# Autodesk Inventor assembly: ASY ДМФ 0100 Барабан
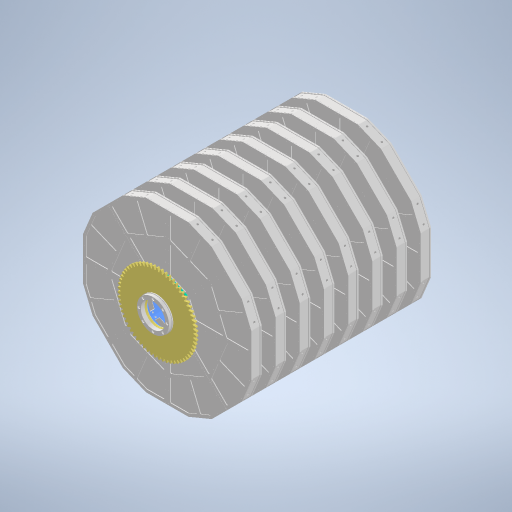
[picture p0: Inventor's stored thumbnail of the model, 512x512]
Saved by Autodesk Inventor 2024.2 (Build 282272000, 272)
## iProperties
Created: 2024-04-28
Part Number: ASY ДМФ 0100 Барабан
Document SubType Name: Assembly
Designer: pokla
Author: pokla
## Documents named in this file (13)
- C:\Users\pokla\Documents\Inventor\ДФО\ДМФ\DMF-Disk-Micro-Filter\ASY ДМФ 0100 Барабан.iam
- C:\Users\pokla\Documents\Inventor\ДФО\ДМФ\DMF-Disk-Micro-Filter\ДМФ 01 21 Барабан торец НОС.ipt
- C:\Users\pokla\Documents\Inventor\ДФО\ДМФ\DMF-Disk-Micro-Filter\ДМФ 01 13 Барабан Лист лев брт.ipt
- C:\Users\pokla\Documents\Inventor\ДФО\ДМФ\DMF-Disk-Micro-Filter\ДМФ 01 14 Барабан Лист прав брт.ipt
- C:\Users\pokla\Documents\Inventor\ДФО\ДМФ\DMF-Disk-Micro-Filter\ДМФ 01 31 Барабан Опорное кольцо НОС.ipt
- C:\Users\pokla\Documents\Inventor\ДФО\ДМФ\DMF-Disk-Micro-Filter\ДМФ 01 17 опора крышки.ipt
- C:\Users\pokla\Documents\Inventor\ДФО\ДМФ\DMF-Disk-Micro-Filter\ДМС 000 размеры.ipt
- C:\Users\pokla\Documents\Inventor\ДФО\ДМФ\DMF-Disk-Micro-Filter\ДМФ 01 41 Шестерня ведомая.ipt
- C:\Users\pokla\Documents\Inventor\ДФО\ДМФ\DMF-Disk-Micro-Filter\ДМФ 01 12 Барабан усилитель.ipt
- C:\Users\pokla\Documents\Inventor\ДФО\ДМФ\DMF-Disk-Micro-Filter\ASY ДМФ 010 крышка.iam
- C:\Users\pokla\Documents\Inventor\ДФО\ДМФ\DMF-Disk-Micro-Filter\ДМФ 01 32 Барабан Опорное кольцо КОРМА.ipt
- C:\Users\pokla\Documents\Inventor\ДФО\ДМФ\DMF-Disk-Micro-Filter\ДМФ 01 22 Барабан торец КОРМА.ipt
- C:\Users\pokla\Documents\Inventor\ДФО\ДМФ\DMF-Disk-Micro-Filter\ASY фильтр пакет.iam
## Components (67 placed, 12 different names)
1. ДМС 000 размеры:1
2. ДМФ 01 21 Барабан торец НОС:2 — Mate:15, Flush:8, Flush:9, Flush:10, Flush:11, Mate:16, Mate:17, Rigid:19, Mate:19, Flush:14, Mate:21, Flush:15, Flush:16, Flush:17, Mate:23
3. ДМФ 01 31 Барабан Опорное кольцо НОС:1 — Rotational:1
4. ДМФ 01 32 Барабан Опорное кольцо КОРМА:1 — Mate:14, Rigid:18
5. ДМФ 01 22 Барабан торец КОРМА:1 — Rigid:18, Flush:12, Flush:13, Mate:18
6. ДМФ 01 13 Барабан Лист лев брт:1 — Mate:12, Flush:7, Flush:10, Flush:11, Mate:16, Flush:13, Mate:18, Mate:20
7. ДМФ 01 14 Барабан Лист прав брт:1 — Mate:11, Flush:8, Flush:9, Mate:17, Flush:12, Mate:22
8. ДМФ 01 17 опора крышки:1 — Mate:21, Flush:15, Mate:22
9. ДМФ 01 17 опора крышки:2 — Mate:19, Mate:20, Flush:14
10. ДМС 105 Шестерня ведомая:1 — Rigid:19, Rotational:1
11. ASY ДМФ 010 крышка:1 [sub-assembly] — Flush:16, Flush:17, Mate:23
12. ДМФ 01 12 Барабан усилитель:4 — Rigid:10
13. ДМФ 01 12 Барабан усилитель:1 — Rigid:8
14. ДМФ 01 12 Барабан усилитель:5 — Rigid:10, Rigid:11, Rigid:14
15. ДМФ 01 12 Барабан усилитель:2 — Rigid:8, Rigid:9, Rigid:14
16. ДМФ 01 12 Барабан усилитель:3 — Rigid:9, Mate:12
17. ДМФ 01 12 Барабан усилитель:6 — Rigid:11
18. ДМФ 01 12 Барабан усилитель:7
19. ДМФ 01 12 Барабан усилитель:8
20. ДМФ 01 12 Барабан усилитель:21
21. ДМФ 01 12 Барабан усилитель:28
22. ДМФ 01 12 Барабан усилитель:35
23. ДМФ 01 12 Барабан усилитель:42
24. ДМФ 01 12 Барабан усилитель:9
25. ДМФ 01 12 Барабан усилитель:10
26. ДМФ 01 12 Барабан усилитель:22
27. ДМФ 01 12 Барабан усилитель:29
28. ДМФ 01 12 Барабан усилитель:36
29. ДМФ 01 12 Барабан усилитель:43
30. ДМФ 01 12 Барабан усилитель:11
31. ДМФ 01 12 Барабан усилитель:12
32. ДМФ 01 12 Барабан усилитель:23
33. ДМФ 01 12 Барабан усилитель:30
34. ДМФ 01 12 Барабан усилитель:37
35. ДМФ 01 12 Барабан усилитель:44
36. ДМФ 01 12 Барабан усилитель:13
37. ДМФ 01 12 Барабан усилитель:14
38. ДМФ 01 12 Барабан усилитель:24
39. ДМФ 01 12 Барабан усилитель:31
40. ДМФ 01 12 Барабан усилитель:38
41. ДМФ 01 12 Барабан усилитель:45
42. ДМФ 01 12 Барабан усилитель:15
43. ДМФ 01 12 Барабан усилитель:16
44. ДМФ 01 12 Барабан усилитель:25
45. ДМФ 01 12 Барабан усилитель:32
46. ДМФ 01 12 Барабан усилитель:39
47. ДМФ 01 12 Барабан усилитель:46
48. ДМФ 01 12 Барабан усилитель:17
49. ДМФ 01 12 Барабан усилитель:18
50. ДМФ 01 12 Барабан усилитель:26
51. ДМФ 01 12 Барабан усилитель:33
52. ДМФ 01 12 Барабан усилитель:40
53. ДМФ 01 12 Барабан усилитель:47
54. ДМФ 01 12 Барабан усилитель:19 — Mate:11
55. ДМФ 01 12 Барабан усилитель:20
56. ДМФ 01 12 Барабан усилитель:27
57. ДМФ 01 12 Барабан усилитель:34
58. ДМФ 01 12 Барабан усилитель:41
59. ДМФ 01 12 Барабан усилитель:48 — Flush:7, Mate:26
60. ASY фильтр пакет:1 [sub-assembly] — Mate:24, Mate:25, Mate:26
61. ASY фильтр пакет:2 [sub-assembly]
62. ASY фильтр пакет:3 [sub-assembly]
63. ASY фильтр пакет:4 [sub-assembly]
64. ASY фильтр пакет:5 [sub-assembly]
65. ASY фильтр пакет:6 [sub-assembly]
66. ASY фильтр пакет:7 [sub-assembly]
67. ASY фильтр пакет:8 [sub-assembly]
## Component patterns: (8 elements, first: ДМФ 01 12 Барабан усилитель:4 + ДМФ 01 12 Барабан усилитель:1 + ДМФ 01 12 Барабан усилитель:5 + ДМФ 01 12 Барабан усилитель:2 + ДМФ 01 12 Барабан усилитель:3 + ДМФ 01 12 Барабан усилитель:6), (8 elements, first: ASY фильтр пакет:1)
## Relationships (35: Mate 15, Flush 11, WeldJoint 8, RevoluteJoint 1)
- Rigid:8 [WeldJoint]: ДМФ 01 12 Барабан усилитель:1 ↔ ДМФ 01 12 Барабан усилитель:2
- Rigid:9 [WeldJoint]: ДМФ 01 12 Барабан усилитель:2 ↔ ДМФ 01 12 Барабан усилитель:3
- Rigid:10 [WeldJoint]: ДМФ 01 12 Барабан усилитель:4 ↔ ДМФ 01 12 Барабан усилитель:5
- Rigid:11 [WeldJoint]: ДМФ 01 12 Барабан усилитель:5 ↔ ДМФ 01 12 Барабан усилитель:6
- Rigid:14 [WeldJoint] (108 mm): ДМФ 01 12 Барабан усилитель:5 ↔ ДМФ 01 12 Барабан усилитель:2
- Mate:11: ДМФ 01 14 Барабан Лист прав брт:1 ↔ ДМФ 01 12 Барабан усилитель:19
- Mate:12: ДМФ 01 13 Барабан Лист лев брт:1 ↔ ДМФ 01 12 Барабан усилитель:3
- Flush:7 (29 mm): ДМФ 01 13 Барабан Лист лев брт:1 ↔ ДМФ 01 12 Барабан усилитель:48
- [WeldJoint] (5 mm): ASY ДМФ 010 крышка:1 ↔ ASY фильтр пакет:1
- Mate:14: ДМФ 01 32 Барабан Опорное кольцо КОРМА:1
- Rigid:18 [WeldJoint]: ДМФ 01 32 Барабан Опорное кольцо КОРМА:1 ↔ ДМФ 01 22 Барабан торец КОРМА:1
- Mate:15: ДМФ 01 21 Барабан торец НОС:2
- Flush:8: ДМФ 01 21 Барабан торец НОС:2 ↔ ДМФ 01 14 Барабан Лист прав брт:1
- Flush:9: ДМФ 01 21 Барабан торец НОС:2 ↔ ДМФ 01 14 Барабан Лист прав брт:1
- Flush:10: ДМФ 01 21 Барабан торец НОС:2 ↔ ДМФ 01 13 Барабан Лист лев брт:1
- Flush:11: ДМФ 01 21 Барабан торец НОС:2 ↔ ДМФ 01 13 Барабан Лист лев брт:1
- Mate:16: ДМФ 01 21 Барабан торец НОС:2 ↔ ДМФ 01 13 Барабан Лист лев брт:1
- Mate:17: ДМФ 01 21 Барабан торец НОС:2 ↔ ДМФ 01 14 Барабан Лист прав брт:1
- Flush:12: ДМФ 01 22 Барабан торец КОРМА:1 ↔ ДМФ 01 14 Барабан Лист прав брт:1
- Flush:13: ДМФ 01 22 Барабан торец КОРМА:1 ↔ ДМФ 01 13 Барабан Лист лев брт:1
- Mate:18: ДМФ 01 22 Барабан торец КОРМА:1 ↔ ДМФ 01 13 Барабан Лист лев брт:1
- Rigid:19 [WeldJoint]: ДМФ 01 21 Барабан торец НОС:2 ↔ ДМС 105 Шестерня ведомая:1
- Rotational:1 [RevoluteJoint]: ДМФ 01 31 Барабан Опорное кольцо НОС:1 ↔ ДМС 105 Шестерня ведомая:1
- Mate:19: ДМФ 01 21 Барабан торец НОС:2 ↔ ДМФ 01 17 опора крышки:2
- Mate:20: ДМФ 01 13 Барабан Лист лев брт:1 ↔ ДМФ 01 17 опора крышки:2
- Flush:14 (2 mm): ДМФ 01 21 Барабан торец НОС:2 ↔ ДМФ 01 17 опора крышки:2
- Mate:21: ДМФ 01 21 Барабан торец НОС:2 ↔ ДМФ 01 17 опора крышки:1
- Flush:15 (-2 mm): ДМФ 01 21 Барабан торец НОС:2 ↔ ДМФ 01 17 опора крышки:1
- Mate:22: ДМФ 01 14 Барабан Лист прав брт:1 ↔ ДМФ 01 17 опора крышки:1
- Flush:16: ДМФ 01 21 Барабан торец НОС:2 ↔ ASY ДМФ 010 крышка:1
- Flush:17: ДМФ 01 21 Барабан торец НОС:2 ↔ ASY ДМФ 010 крышка:1
- Mate:23: ДМФ 01 21 Барабан торец НОС:2 ↔ ASY ДМФ 010 крышка:1
- Mate:24: ASY фильтр пакет:1
- Mate:25: ASY фильтр пакет:1
- Mate:26: ДМФ 01 12 Барабан усилитель:48 ↔ ASY фильтр пакет:1
